# Autodesk Inventor assembly: Latest Assembly
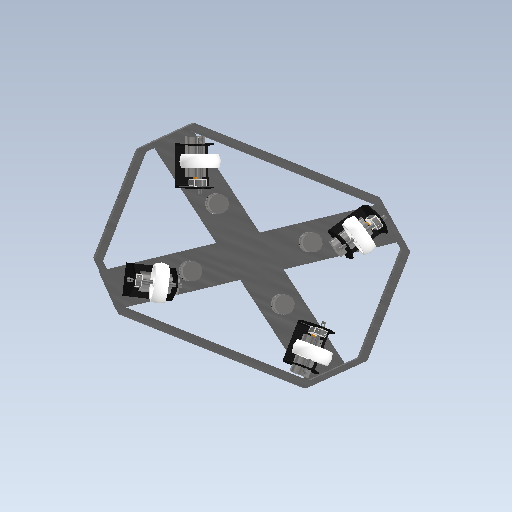
[picture p0: Inventor's stored thumbnail of the model, 512x512]
Saved by Autodesk Inventor 2020 (Build 240168000, 168)
## iProperties
Created: 2022-07-18
Part Number: Latest Assembly
Document SubType Name: Assembly
Designer: karimi2
Author: karimi2
## Documents named in this file (8)
- C:\Users\karimi2\Documents\PROJECT\src\Latest Assembly.iam
- C:\Users\karimi2\Documents\PROJECT\src\Wheel Assembly.iam
- C:\Users\karimi2\Documents\PROJECT\src\New Chassis.ipt
- C:\Users\karimi2\Documents\PROJECT\src\GearedDCmotor.ipt
- C:\Users\karimi2\Documents\PROJECT\src\Latest Assembly\Design Accelerator\Synchronous Belts Transmission3.iam
- C:\Users\karimi2\Documents\PROJECT\src\Latest Assembly\Design Accelerator\Synchronous Belts Transmission4.iam
- C:\Users\karimi2\Documents\PROJECT\src\Latest Assembly\Design Accelerator\Synchronous Belts Transmission5.iam
- C:\Users\karimi2\Documents\PROJECT\src\Latest Assembly\Design Accelerator\Synchronous Belts Transmission6.iam
## Components (13 placed, 4 different names)
1. Wheel Assembly:1 [sub-assembly] — Mate:1, Rotational:1, Mate:8, Rigid:4
2. New Chassis:1 — Mate:1, Rotational:1, Mate:2, Rigid:1, Mate:3, Rotational:2, Mate:4, Rigid:2, Mate:12, Rotational:3, Mate:13, Rigid:6, Mate:16, Rotational:4, Mate:17, Rigid:8
3. GearedDCmotor:1 — Mate:2, Rigid:1, Mate:9
4. Wheel Assembly:2 [sub-assembly] — Mate:3, Rotational:2, Mate:11, Rigid:5
5. GearedDCmotor:4 — Mate:4, Rigid:2, Mate:10
6. Synchronous Belts Transmission:3 [sub-assembly] — Mate:8, Mate:9, Rigid:4
7. Synchronous Belts Transmission:4 [sub-assembly] — Mate:10, Mate:11, Rigid:5
8. Wheel Assembly:3 [sub-assembly] — Mate:12, Rotational:3, Mate:15, Rigid:7
9. GearedDCmotor:5 — Mate:13, Rigid:6, Mate:14
10. Synchronous Belts Transmission:5 [sub-assembly] — Mate:14, Mate:15, Rigid:7
11. Wheel Assembly:4 [sub-assembly] — Mate:16, Rotational:4, Mate:19, Rigid:9
12. GearedDCmotor:6 — Mate:17, Rigid:8, Mate:18
13. Synchronous Belts Transmission:6 [sub-assembly] — Mate:18, Mate:19, Rigid:9
## Relationships (28: Mate 16, WeldJoint 8, RevoluteJoint 4)
- Mate:1: Wheel Assembly:1 ↔ New Chassis:1
- Rotational:1 [RevoluteJoint] (-5 mm): Wheel Assembly:1 ↔ New Chassis:1
- Mate:2: New Chassis:1 ↔ GearedDCmotor:1
- Rigid:1 [WeldJoint]: New Chassis:1 ↔ GearedDCmotor:1
- Mate:3: New Chassis:1 ↔ Wheel Assembly:2
- Rotational:2 [RevoluteJoint] (-5 mm): New Chassis:1 ↔ Wheel Assembly:2
- Mate:4: New Chassis:1 ↔ GearedDCmotor:4
- Rigid:2 [WeldJoint] (-6 mm): New Chassis:1 ↔ GearedDCmotor:4
- Mate:8: Wheel Assembly:1 ↔ Synchronous Belts Transmission:3
- Mate:9: GearedDCmotor:1 ↔ Synchronous Belts Transmission:3
- Rigid:4 [WeldJoint] (-2 mm): Wheel Assembly:1 ↔ Synchronous Belts Transmission:3
- Mate:10: GearedDCmotor:4 ↔ Synchronous Belts Transmission:4
- Mate:11: Wheel Assembly:2 ↔ Synchronous Belts Transmission:4
- Rigid:5 [WeldJoint] (-2 mm): Wheel Assembly:2 ↔ Synchronous Belts Transmission:4
- Mate:12: New Chassis:1 ↔ Wheel Assembly:3
- Rotational:3 [RevoluteJoint] (-5 mm): New Chassis:1 ↔ Wheel Assembly:3
- Mate:13: New Chassis:1 ↔ GearedDCmotor:5
- Rigid:6 [WeldJoint] (-6 mm): New Chassis:1 ↔ GearedDCmotor:5
- Mate:14: GearedDCmotor:5 ↔ Synchronous Belts Transmission:5
- Mate:15: Wheel Assembly:3 ↔ Synchronous Belts Transmission:5
- Rigid:7 [WeldJoint] (-2 mm): Wheel Assembly:3 ↔ Synchronous Belts Transmission:5
- Mate:16: New Chassis:1 ↔ Wheel Assembly:4
- Rotational:4 [RevoluteJoint] (-5 mm): New Chassis:1 ↔ Wheel Assembly:4
- Mate:17: New Chassis:1 ↔ GearedDCmotor:6
- Rigid:8 [WeldJoint] (-6 mm): New Chassis:1 ↔ GearedDCmotor:6
- Mate:18: GearedDCmotor:6 ↔ Synchronous Belts Transmission:6
- Mate:19: Wheel Assembly:4 ↔ Synchronous Belts Transmission:6
- Rigid:9 [WeldJoint] (-2 mm): Wheel Assembly:4 ↔ Synchronous Belts Transmission:6
